# Autodesk Inventor assembly: Shock_Absorber
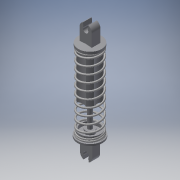
[picture p0: Inventor's stored thumbnail of the model, 180x180]
Saved by Autodesk Inventor 2019 (Build 230136000, 136)
## iProperties
Created: 2019-03-03
Part Number: Shock_Absorber
Document SubType Name: Assembly
Designer: alarr
Author: alarr
## Documents named in this file (4)
- C:\Users\alarr\OneDrive\Documents\Inventor\Mr.Green\Shock_Absorber.iam
- C:\Users\alarr\OneDrive\Documents\Inventor\Mr.Green\Bottom.ipt
- C:\Users\alarr\OneDrive\Documents\Inventor\Mr.Green\Top.ipt
- C:\Users\alarr\OneDrive\Documents\Inventor\Mr.Green\Shock_Absorber\Design Accelerator\Compress Spring1.iam
## Components (3 placed, 3 different names)
1. Bottom:1 — Mate:1, Angle:1, Flush:1
2. Top:1 — Mate:1, Angle:1, Mate:4
3. Compress Spring:1 [sub-assembly] — Mate:3, Flush:1, Mate:4
## Relationships (5: Mate 3, Angle 1, Flush 1)
- Mate:1: Bottom:1 ↔ Top:1
- Angle:1 (0 deg): Bottom:1 ↔ Top:1
- Mate:3: Compress Spring:1
- Flush:1: Bottom:1 ↔ Compress Spring:1
- Mate:4: Top:1 ↔ Compress Spring:1
